# Autodesk Inventor assembly: Pinky_Assembly_01
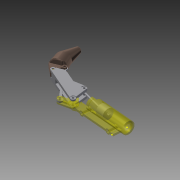
[picture p0: Inventor's stored thumbnail of the model, 180x180]
Saved by Autodesk Inventor 2015 (Build 190159000, 159)
## iProperties
Created: 2016-09-17
Part Number: Pinky_Assembly_01
Document SubType Name: Assembly
Designer: Neelotpal Nag
Author: Neelotpal Nag
## Documents named in this file (7)
- D:\NEEL BACKUP\DISA 2016\Fingers 1\Pinky\Pinky_Assembly_01.iam
- D:\NEEL BACKUP\DISA 2016\Fingers 1\Pinky\Cylinder_10.5mm.ipt
- D:\NEEL BACKUP\DISA 2016\Fingers 1\Pinky\Restrain_Pin_Pinky_1.ipt
- D:\NEEL BACKUP\DISA 2016\Fingers 1\Pinky\Shaft_Piston.ipt
- D:\NEEL BACKUP\DISA 2016\Fingers 1\Pinky\Base_Cylinder_Pinky_11mm.ipt
- D:\NEEL BACKUP\DISA 2016\Fingers 1\Pinky\Pinky_Lower_main_1.ipt
- D:\NEEL BACKUP\DISA 2016\Fingers 1\Pinky\Pinky_Upper_main_2.ipt
## Components (6 placed, 6 different names)
1. Cylinder_10.5mm:1 — Mate:1, Angle:1, Mate:9, Mate:10
2. Restrain_Pin_Pinky_1:1 — Mate:6, Mate:7, Mate:8
3. Shaft_Piston:1 — Mate:9, Mate:10, Mate:11
4. Base_Cylinder_Pinky_11mm:1 — Mate:1, Angle:1, Mate:2, Mate:3, Mate:7, Mate:8
5. Pinky_Lower_main_1:1 — Mate:2, Mate:3, Mate:4, Mate:5, Mate:11
6. Pinky_Upper_main_2:1 — Mate:4, Mate:5, Mate:6
## Relationships (12: Mate 11, Angle 1)
- Mate:1: Cylinder_10.5mm:1 ↔ Base_Cylinder_Pinky_11mm:1
- Angle:1 (0 deg): Cylinder_10.5mm:1 ↔ Base_Cylinder_Pinky_11mm:1
- Mate:2: Base_Cylinder_Pinky_11mm:1 ↔ Pinky_Lower_main_1:1
- Mate:3: Base_Cylinder_Pinky_11mm:1 ↔ Pinky_Lower_main_1:1
- Mate:4: Pinky_Lower_main_1:1 ↔ Pinky_Upper_main_2:1
- Mate:5: Pinky_Lower_main_1:1 ↔ Pinky_Upper_main_2:1
- Mate:6: Restrain_Pin_Pinky_1:1 ↔ Pinky_Upper_main_2:1
- Mate:7: Restrain_Pin_Pinky_1:1 ↔ Base_Cylinder_Pinky_11mm:1
- Mate:8 (-3 mm): Restrain_Pin_Pinky_1:1 ↔ Base_Cylinder_Pinky_11mm:1
- Mate:9: Cylinder_10.5mm:1 ↔ Shaft_Piston:1
- Mate:10: Cylinder_10.5mm:1 ↔ Shaft_Piston:1
- Mate:11: Shaft_Piston:1 ↔ Pinky_Lower_main_1:1
